# Autodesk Inventor assembly: reductor
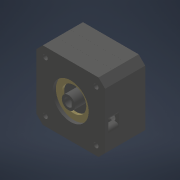
[picture p0: Inventor's stored thumbnail of the model, 180x180]
Saved by Autodesk Inventor 2022 (Build 260153070, 153G)
## iProperties
Created: 2021-11-20
Part Number: reductor
Document SubType Name: Assembly
Designer: Teo
Mass: 53.2083 g
Surface Area: 276.75 cm^2
Volume: 30.913 cm^3
Density: 1.72123 g/cm^3
Title: Predstavitev sklopa
Author: Teo
## Documents named in this file (12)
- D:\Zaključna\Roka\Priloge\IPT_files\Assemblies\reductor.iam
- D:\Zaključna\Roka\Priloge\IPT_files\Cicloidal_gear\Stator_encoder_lite.ipt
- D:\Zaključna\Roka\Priloge\IPT_files\Cicloidal_gear\Center_encoder_lite.ipt
- D:\Zaključna\Roka\Priloge\IPT_files\Cicloidal_gear\Excenter_lite.ipt
- D:\Zaključna\Roka\Priloge\IPT_files\Cicloidal_gear\Stator_lite.ipt
- D:\Zaključna\Roka\Priloge\IPT_files\Cicloidal_gear\Disk_lite.ipt
- C:\Users\Teo\Documents\Inventor\Content Center Files\R2022\en-US\DIN 625 - T1\DIN 625 T1 - 619_8 - 8 x 19 x 6.ipt
- D:\Zaključna\Roka\Priloge\IPT_files\Cicloidal_gear\Center_lite.ipt
- D:\Zaključna\Roka\Priloge\IPT_files\Cicloidal_gear\Rotor_lite.ipt
- D:\Zaključna\Roka\Priloge\IPT_files\Cicloidal_gear\Housing_lite.ipt
- D:\Zaključna\Roka\Priloge\PCB\Board.ipt
- D:\Zaključna\Roka\Priloge\IPT_files\Magnet.ipt
## Components (12 placed, 11 different names)
1. Stator_encoder_lite:1 — Flush:1, Mate:1, Mate:4, Mate:5, Mate:6, Mate:24, Mate:25, Mate:26
2. Center_encoder_lite:1 — Flush:1, Mate:1, Flush:2, Mate:12, Mate:14, Mate:27, Flush:4
3. Excenter_lite:1 — Flush:2, Mate:7, Mate:11, Mate:12, Mate:14, Mate:15, Mate:16, Flush:3, Rotation:1
4. Stator_lite:1 — Mate:4, Mate:5, Mate:6, Mate:20, Mate:21, Mate:22, Mate:23
5. Disk_lite:1 — Mate:10, Mate:13, Rotation:1, Rotation:2
6. DIN 625 - T1 619/8 - 8 x 19 x 6:1 — Mate:7, Mate:10, Mate:11, Mate:13
7. Center_lite:1 — Mate:15, Mate:16, Flush:3, Mate:17, Mate:18
8. DIN 625 - T1 619/8 - 8 x 19 x 6:2 — Mate:17, Mate:18, Mate:19
9. Rotor_lite:1 — Mate:19, Mate:20, Rotation:2
10. Housing_lite:1 — Mate:21, Mate:22, Mate:23
11. Board:1 — Mate:24, Mate:25, Mate:26
12. Magnet:1 — Mate:27, Flush:4
## Relationships (29: Mate 23, Flush 4, RelateRotation 2)
- Flush:1 (-1.4 mm): Stator_encoder_lite:1 ↔ Center_encoder_lite:1
- Mate:1: Stator_encoder_lite:1 ↔ Center_encoder_lite:1
- Flush:2: Center_encoder_lite:1 ↔ Excenter_lite:1
- Mate:4: Stator_encoder_lite:1 ↔ Stator_lite:1
- Mate:5: Stator_encoder_lite:1 ↔ Stator_lite:1
- Mate:6: Stator_encoder_lite:1 ↔ Stator_lite:1
- Mate:7: Excenter_lite:1 ↔ DIN 625 - T1 619/8 - 8 x 19 x 6:1
- Mate:10: Disk_lite:1 ↔ DIN 625 - T1 619/8 - 8 x 19 x 6:1
- Mate:11: Excenter_lite:1 ↔ DIN 625 - T1 619/8 - 8 x 19 x 6:1
- Mate:12: Center_encoder_lite:1 ↔ Excenter_lite:1
- Mate:13: Disk_lite:1 ↔ DIN 625 - T1 619/8 - 8 x 19 x 6:1
- Mate:14: Center_encoder_lite:1 ↔ Excenter_lite:1
- Mate:15: Excenter_lite:1 ↔ Center_lite:1
- Mate:16: Excenter_lite:1 ↔ Center_lite:1
- Flush:3: Excenter_lite:1 ↔ Center_lite:1
- Mate:17: Center_lite:1 ↔ DIN 625 - T1 619/8 - 8 x 19 x 6:2
- Mate:18: Center_lite:1 ↔ DIN 625 - T1 619/8 - 8 x 19 x 6:2
- Mate:19: DIN 625 - T1 619/8 - 8 x 19 x 6:2 ↔ Rotor_lite:1
- Mate:20: Stator_lite:1 ↔ Rotor_lite:1
- Mate:21: Stator_lite:1 ↔ Housing_lite:1
- Mate:22: Stator_lite:1 ↔ Housing_lite:1
- Mate:23: Stator_lite:1 ↔ Housing_lite:1
- Rotation:1 [RelateRotation] (11 ul): Excenter_lite:1 ↔ Disk_lite:1
- Rotation:2 [RelateRotation] (0.3333 ul): Disk_lite:1 ↔ Rotor_lite:1
- Mate:24: Stator_encoder_lite:1 ↔ Board:1
- Mate:25: Stator_encoder_lite:1 ↔ Board:1
- Mate:26: Stator_encoder_lite:1 ↔ Board:1
- Mate:27: Center_encoder_lite:1 ↔ Magnet:1
- Flush:4: Center_encoder_lite:1 ↔ Magnet:1
